# Autodesk Inventor assembly: Xaxis_VarB
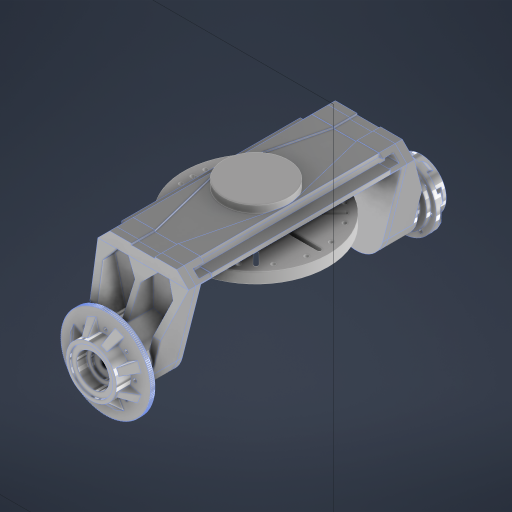
[picture p0: Inventor's stored thumbnail of the model, 512x512]
Saved by Autodesk Inventor 2024 (Build 280153000, 153)
## iProperties
Created: 2023-03-08
Part Number: Xaxis_VarB
Document SubType Name: Assembly
Designer: KirikDK
Mass: 30913.1 g
Surface Area: 20634.3 cm^2
Volume: 14365 cm^3
Density: 2.15197 g/cm^3
Author: KirikDK
## Documents named in this file (11)
- C:\Users\KirikDK\Documents\Stanok2023\Aaxis_Ass.iam
- C:\Users\KirikDK\Documents\Stanok2023\A_axisShesterna.ipt
- C:\Users\KirikDK\Documents\Stanok2023\A_axisFlanec.ipt
- C:\Users\KirikDK\Documents\Stanok2023\KrovatkaShatunFlanec.ipt
- C:\Users\KirikDK\Documents\Stanok2023\KrovatkaShatunPods.ipt
- C:\Users\KirikDK\Documents\Stanok2023\A_axisZagluska.ipt
- C:\Users\KirikDK\Documents\Stanok2023\A_AxisKrovatka.ipt
- C:\Users\KirikDK\Documents\Stanok2023\Osnova.ipt
- C:\Users\KirikDK\Documents\Stanok2023\OsnovaNiz.ipt
- C:\Users\KirikDK\Documents\Stanok2023\B_axisColeso.ipt
- C:\Users\KirikDK\Documents\Stanok2023\BaxisStol.ipt
## Components (13 placed, 10 different names)
1. A_axisShesterna:1 — Mate:83, Mate:84
2. A_axisFlanec:1 — Mate:61
3. KrovatkaShatunFlanec:3 — Mate:81, Flush:17, Flush:19
4. KrovatkaShatunPods:2 — Mate:59, Mate:60, Mate:76, Flush:19
5. A_axisZagluska:2 — Mate:59, Mate:60, Mate:61
6. A_AxisKrovatka:1 — Mate:78, Mate:82, Mate:85, Flush:21
7. KrovatkaShatunFlanec:6 — Mate:80, Flush:18, Flush:20, Mate:86
8. KrovatkaShatunPods:5 — Mate:76, Flush:20
9. A_axisZagluska:4 — Mate:83, Mate:84
10. Osnova:1 — Mate:78, Mate:80, Mate:81, Flush:17, Flush:18, Mate:82, Mate:89, Mate:90
11. OsnovaNiz:1 — Mate:85, Flush:21, Mate:86, Mate:87, Mate:88
12. B_axisColeso:2 — Mate:87, Mate:88
13. BaxisStol:1 — Mate:89, Mate:90
## Relationships (27: Mate 20, Flush 7)
- [Mate]: KrovatkaShatunFlanec:3 ↔ KrovatkaShatunPods:2
- [Flush]: KrovatkaShatunFlanec:3 ↔ KrovatkaShatunPods:2
- Mate:59: KrovatkaShatunPods:2 ↔ A_axisZagluska:2
- Mate:60: KrovatkaShatunPods:2 ↔ A_axisZagluska:2
- Mate:61: A_axisFlanec:1 ↔ A_axisZagluska:2
- [Mate]: KrovatkaShatunFlanec:6 ↔ KrovatkaShatunPods:5
- [Flush]: KrovatkaShatunFlanec:6 ↔ KrovatkaShatunPods:5
- [Mate]: KrovatkaShatunPods:5 ↔ A_axisZagluska:4
- [Mate]: KrovatkaShatunPods:5 ↔ A_axisZagluska:4
- Mate:76: KrovatkaShatunPods:2 ↔ KrovatkaShatunPods:5
- Mate:78: A_AxisKrovatka:1 ↔ Osnova:1
- Mate:80: KrovatkaShatunFlanec:6 ↔ Osnova:1
- Mate:81: KrovatkaShatunFlanec:3 ↔ Osnova:1
- Flush:17: KrovatkaShatunFlanec:3 ↔ Osnova:1
- Flush:18: KrovatkaShatunFlanec:6 ↔ Osnova:1
- Mate:82: A_AxisKrovatka:1 ↔ Osnova:1
- Flush:19: KrovatkaShatunFlanec:3 ↔ KrovatkaShatunPods:2
- Flush:20: KrovatkaShatunFlanec:6 ↔ KrovatkaShatunPods:5
- Mate:83: A_axisShesterna:1 ↔ A_axisZagluska:4
- Mate:84: A_axisShesterna:1 ↔ A_axisZagluska:4
- Mate:85: A_AxisKrovatka:1 ↔ OsnovaNiz:1
- Flush:21: A_AxisKrovatka:1 ↔ OsnovaNiz:1
- Mate:86: KrovatkaShatunFlanec:6 ↔ OsnovaNiz:1
- Mate:87: OsnovaNiz:1 ↔ B_axisColeso:2
- Mate:88: OsnovaNiz:1 ↔ B_axisColeso:2
- Mate:89: Osnova:1 ↔ BaxisStol:1
- Mate:90: Osnova:1 ↔ BaxisStol:1
## Named parameters: d96_d93 = 0 mm, d97_d94 = 0 mm, d123_d116_d104 = 0 mm, d124_d117_d105 = 0 mm, d125_d118_d101_d93 = 0 mm, d126_d119_d102_d94 = 0 mm
